# Autodesk Inventor assembly: railBearing
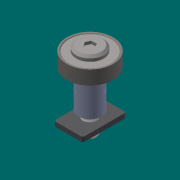
[picture p0: Inventor's stored thumbnail of the model, 180x180]
Saved by Autodesk Inventor 2016 SP1 (Build 200210100, 210)
## iProperties
Created: 2016-03-13
Part Number: railBearing
Document SubType Name: Assembly
Designer: sawaiz
Author: sawaiz
## Documents named in this file (5)
- C:\Users\sawaiz\OneDrive\projects\modularRichFrame\rail\railBearing.iam
- C:\Users\sawaiz\OneDrive\projects\modularRichFrame\hardware\625BallBearing.ipt
- C:\Users\sawaiz\OneDrive\projects\modularRichFrame\hardware\0.25inSpacer.ipt
- C:\Users\sawaiz\oneDrive\projects\modularRichFrame\hardware\m5TNut.ipt
- C:\Users\sawaiz\OneDrive\projects\modularRichFrame\hardware\m5x25LowProfile.ipt
## Components (5 placed, 4 different names)
1. 625BallBearing:1 — Mate:1, Mate:3, Mate:5, Mate:8
2. 0.25inSpacer:1 — Mate:1, Mate:6, Mate:7, Mate:9
3. m5TNut:1 — Mate:4, Mate:6
4. m5x25LowProfile:1 — Mate:3, Mate:4, Mate:5
5. 0.25inSpacer:2 — Mate:7, Mate:8, Mate:9
## Relationships (8: Mate 8)
- Mate:1: 625BallBearing:1 ↔ 0.25inSpacer:1
- Mate:3: 625BallBearing:1 ↔ m5x25LowProfile:1
- Mate:4: m5TNut:1 ↔ m5x25LowProfile:1
- Mate:5: 625BallBearing:1 ↔ m5x25LowProfile:1
- Mate:6 (2 mm): 0.25inSpacer:1 ↔ m5TNut:1
- Mate:7: 0.25inSpacer:1 ↔ 0.25inSpacer:2
- Mate:8: 625BallBearing:1 ↔ 0.25inSpacer:2
- Mate:9: 0.25inSpacer:1 ↔ 0.25inSpacer:2
